# Autodesk Inventor assembly: Omni Wheel
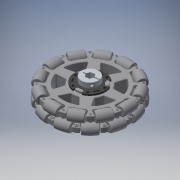
[picture p0: Inventor's stored thumbnail of the model, 180x180]
Saved by Autodesk Inventor 2018 (Build 220112000, 112)
## iProperties
Created: 2018-01-27
Part Number: Omni Wheel
Document SubType Name: Assembly
Designer: maste
Author: maste
## Documents named in this file (5)
- F:\Summer Drive Base V1\Summer Drivebase\Omni Wheel.iam
- F:\Summer Drive Base V1\Summer Drivebase\6_Omni-Directional_Wheel_217-2585.ipt
- F:\Summer Drive Base V1\Summer Drivebase\1_2_Hex_Bore_Aluminum_VersaHub_217-2592.ipt
- F:\Summer Drive Base V1\Summer Drivebase\1_2_Hex_Bore_Plastic_VersaHub_217-4009.ipt
- F:\Summer Drive Base V1\Summer Drivebase\am-1238+Collar+Clamp,+0.5''+Hex+Bore,+Aluminum.iam
## Components (4 placed, 4 different names)
1. 6_Omni-Directional_Wheel_217-2585:1 — Mate:1, Mate:2, Mate:3, Mate:4, Mate:5, Mate:6
2. 1_2_Hex_Bore_Aluminum_VersaHub_217-2592:1 — Mate:4, Mate:5, Mate:6
3. 1_2_Hex_Bore_Plastic_VersaHub_217-4009:1 — Mate:1, Mate:2, Mate:3, Mate:7, Flush:1, Flush:2
4. am-1238+Collar+Clamp,+0.5''+Hex+Bore,+Aluminum:1 [sub-assembly] — Mate:7, Flush:1, Flush:2
## Relationships (9: Mate 7, Flush 2)
- Mate:1: 6_Omni-Directional_Wheel_217-2585:1 ↔ 1_2_Hex_Bore_Plastic_VersaHub_217-4009:1
- Mate:2: 6_Omni-Directional_Wheel_217-2585:1 ↔ 1_2_Hex_Bore_Plastic_VersaHub_217-4009:1
- Mate:3: 6_Omni-Directional_Wheel_217-2585:1 ↔ 1_2_Hex_Bore_Plastic_VersaHub_217-4009:1
- Mate:4: 6_Omni-Directional_Wheel_217-2585:1 ↔ 1_2_Hex_Bore_Aluminum_VersaHub_217-2592:1
- Mate:5: 6_Omni-Directional_Wheel_217-2585:1 ↔ 1_2_Hex_Bore_Aluminum_VersaHub_217-2592:1
- Mate:6: 6_Omni-Directional_Wheel_217-2585:1 ↔ 1_2_Hex_Bore_Aluminum_VersaHub_217-2592:1
- Mate:7: 1_2_Hex_Bore_Plastic_VersaHub_217-4009:1 ↔ am-1238+Collar+Clamp,+0.5''+Hex+Bore,+Aluminum:1
- Flush:1: 1_2_Hex_Bore_Plastic_VersaHub_217-4009:1 ↔ am-1238+Collar+Clamp,+0.5''+Hex+Bore,+Aluminum:1
- Flush:2: 1_2_Hex_Bore_Plastic_VersaHub_217-4009:1 ↔ am-1238+Collar+Clamp,+0.5''+Hex+Bore,+Aluminum:1
